# Autodesk Inventor assembly: Molde_Completo
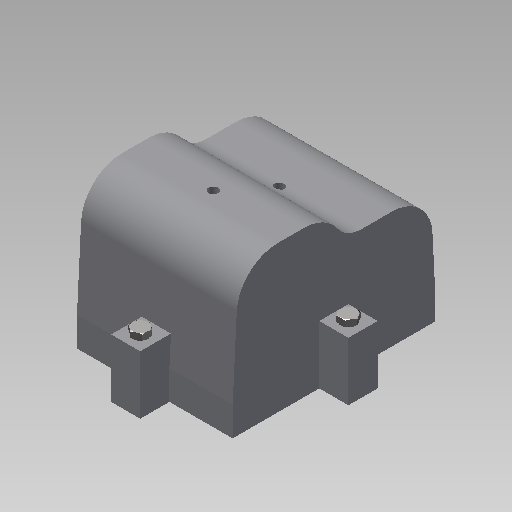
[picture p0: Inventor's stored thumbnail of the model, 512x512]
Saved by Autodesk Inventor 2019 (Build 230136000, 136)
## iProperties
Created: 2019-05-31
Part Number: Molde_Completo
Document SubType Name: Assembly
Designer: Emily Rojas
Author: Emily Rojas
## Documents named in this file (5)
- C:\Users\gusta\Documents\UPB\Diseño\Actividad 5\Molde_Completo.iam
- C:\Users\gusta\Documents\UPB\Diseño\Actividad 5\Molde_Cavidad.ipt
- C:\Users\gusta\Documents\UPB\Diseño\Actividad 5\Molde_Corazon.ipt
- C:\Users\gusta\Documents\UPB\Diseño\Actividad 5\AS 1110 - M5 x 35.ipt
- C:\Users\gusta\Documents\UPB\Diseño\Actividad 5\AS 1112 - M5(2).ipt
## Components (10 placed, 4 different names)
1. Molde_Cavidad:1 — Mate:1, Mate:2, Mate:3, Mate:8, Mate:9, Mate:10, Mate:11, Mate:12, Mate:13, Mate:14, Mate:15
2. Molde_Corazon:1 — Mate:1, Mate:2, Mate:3, Mate:4, Mate:5, Mate:6, Mate:7
3. AS 1110 - Metric M5 x 35:1 — Mate:9, Mate:14, Mate:18
4. AS 1112 (4) - Metric M5:1 — Mate:6, Mate:19
5. AS 1110 - Metric M5 x 35:2 — Mate:10, Mate:15, Mate:16
6. AS 1112 (4) - Metric M5:2 — Mate:4, Mate:18
7. AS 1110 - Metric M5 x 35:3 — Mate:11, Mate:13, Mate:19
8. AS 1112 (4) - Metric M5:3 — Mate:7, Mate:16
9. AS 1110 - Metric M5 x 35:4 — Mate:8, Mate:12, Mate:17
10. AS 1112 (4) - Metric M5:4 — Mate:5, Mate:17
## Relationships (19: Mate 19)
- Mate:1: Molde_Cavidad:1 ↔ Molde_Corazon:1
- Mate:2: Molde_Cavidad:1 ↔ Molde_Corazon:1
- Mate:3: Molde_Cavidad:1 ↔ Molde_Corazon:1
- Mate:4: Molde_Corazon:1 ↔ AS 1112 (4) - Metric M5:2
- Mate:5: Molde_Corazon:1 ↔ AS 1112 (4) - Metric M5:4
- Mate:6: Molde_Corazon:1 ↔ AS 1112 (4) - Metric M5:1
- Mate:7: Molde_Corazon:1 ↔ AS 1112 (4) - Metric M5:3
- Mate:8: Molde_Cavidad:1 ↔ AS 1110 - Metric M5 x 35:4
- Mate:9: Molde_Cavidad:1 ↔ AS 1110 - Metric M5 x 35:1
- Mate:10: Molde_Cavidad:1 ↔ AS 1110 - Metric M5 x 35:2
- Mate:11: Molde_Cavidad:1 ↔ AS 1110 - Metric M5 x 35:3
- Mate:12: Molde_Cavidad:1 ↔ AS 1110 - Metric M5 x 35:4
- Mate:13: Molde_Cavidad:1 ↔ AS 1110 - Metric M5 x 35:3
- Mate:14: Molde_Cavidad:1 ↔ AS 1110 - Metric M5 x 35:1
- Mate:15: Molde_Cavidad:1 ↔ AS 1110 - Metric M5 x 35:2
- Mate:16: AS 1110 - Metric M5 x 35:2 ↔ AS 1112 (4) - Metric M5:3
- Mate:17: AS 1110 - Metric M5 x 35:4 ↔ AS 1112 (4) - Metric M5:4
- Mate:18: AS 1110 - Metric M5 x 35:1 ↔ AS 1112 (4) - Metric M5:2
- Mate:19: AS 1112 (4) - Metric M5:1 ↔ AS 1110 - Metric M5 x 35:3
